# Autodesk Inventor assembly: Roller_Bracket_40mm
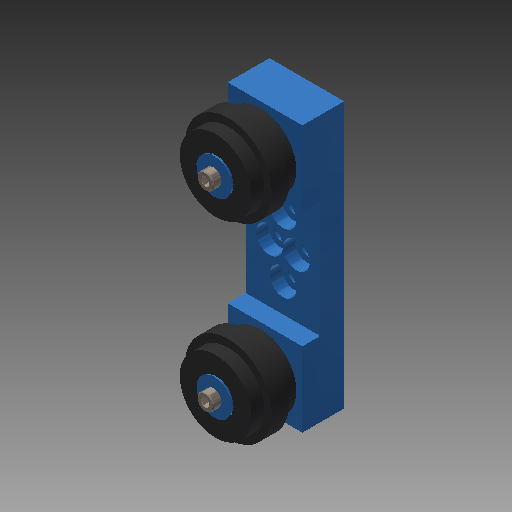
[picture p0: Inventor's stored thumbnail of the model, 512x512]
Saved by Autodesk Inventor 2019.4 (Build 234330000, 330)
## iProperties
Created: 2021-02-01
Part Number: Roller_Bracket_40mm
Document SubType Name: Assembly
Designer: Jorian Brusind
Mass: 44.0669 g
Surface Area: 169.812 cm^2
Volume: 42.4218 cm^3
Density: 1.03878 g/cm^3
Author: Jorian Brusind
## Documents named in this file (6)
- C:\Users\Jorian Brusind\Documents\GitHub\PersonalProjects\HyperRail\Inventor Files\Roller_Bracket_40mm.iam
- C:\Users\Jorian Brusind\Documents\GitHub\PersonalProjects\HyperRail\Inventor Files\RollerWheel.ipt
- C:\Users\Jorian Brusind\Documents\GitHub\PersonalProjects\Inventor Projects\Useful models\Metric bolt\Bolt M3 25mm.ipt
- C:\Users\Jorian Brusind\Documents\GitHub\PersonalProjects\Inventor Projects\Useful models\683ZZBallBearing.ipt
- C:\Users\Jorian Brusind\Documents\GitHub\PersonalProjects\HyperRail\Inventor Files\3mmSpacer.ipt
- C:\Users\Jorian Brusind\Documents\GitHub\PersonalProjects\HyperRail\Inventor Files\Back_Bracket_40mm.ipt
## Components (11 placed, 5 different names)
1. RollerWheel:1 — Mate:3, Flush:3
2. RollerWheel:2 — Mate:6, Flush:2, Mate:17
3. Bolt M3 25mm:1 — Mate:4, Mate:20, Mate:21, Mate:24, Mate:25
4. Bolt M3 25mm:2 — Mate:8, Mate:14, Mate:16, Mate:26
5. 683ZZBallBearing:1 — Mate:3, Mate:4, Flush:3, Mate:22, Mate:23
6. 683ZZBallBearing:2 — Mate:6, Flush:2, Mate:8, Mate:18, Mate:19
7. 3mmSpacer:1 — Mate:14, Mate:16, Mate:18
8. 3mmSpacer:2 — Mate:17, Mate:19, Mate:27
9. 3mmSpacer:3 — Mate:20, Mate:22, Mate:24
10. 3mmSpacer:4 — Mate:21, Mate:23, Mate:28
11. Back_Bracket_40mm:1 — Mate:25, Mate:26, Mate:27, Mate:28
## Relationships (20: Mate 18, Flush 2)
- Mate:3: RollerWheel:1 ↔ 683ZZBallBearing:1
- Mate:4: Bolt M3 25mm:1 ↔ 683ZZBallBearing:1
- Mate:6: RollerWheel:2 ↔ 683ZZBallBearing:2
- Flush:2 (5.5 mm): RollerWheel:2 ↔ 683ZZBallBearing:2
- Mate:8: Bolt M3 25mm:2 ↔ 683ZZBallBearing:2
- Mate:14: Bolt M3 25mm:2 ↔ 3mmSpacer:1
- Mate:16: Bolt M3 25mm:2 ↔ 3mmSpacer:1
- Mate:17: RollerWheel:2 ↔ 3mmSpacer:2
- Mate:18: 683ZZBallBearing:2 ↔ 3mmSpacer:1
- Mate:19: 683ZZBallBearing:2 ↔ 3mmSpacer:2
- Flush:3 (5.5 mm): RollerWheel:1 ↔ 683ZZBallBearing:1
- Mate:20: Bolt M3 25mm:1 ↔ 3mmSpacer:3
- Mate:21: Bolt M3 25mm:1 ↔ 3mmSpacer:4
- Mate:22: 683ZZBallBearing:1 ↔ 3mmSpacer:3
- Mate:23: 683ZZBallBearing:1 ↔ 3mmSpacer:4
- Mate:24: Bolt M3 25mm:1 ↔ 3mmSpacer:3
- Mate:25: Bolt M3 25mm:1 ↔ Back_Bracket_40mm:1
- Mate:26: Bolt M3 25mm:2 ↔ Back_Bracket_40mm:1
- Mate:27 (1 mm): 3mmSpacer:2 ↔ Back_Bracket_40mm:1
- Mate:28 (1 mm): 3mmSpacer:4 ↔ Back_Bracket_40mm:1
